# Autodesk Inventor assembly: Assembly33
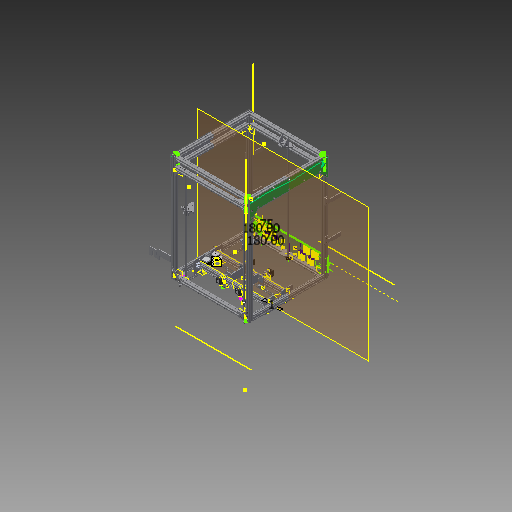
[picture p0: Inventor's stored thumbnail of the model, 512x512]
Saved by Autodesk Inventor 2018 (Build 220112000, 112)
## iProperties
Created: 2016-08-03
Part Number: Assembly33
Document SubType Name: Assembly
Designer: User
Author: User
## Documents named in this file (51)
- C:\Users\Dan\OneDrive\SL-Inventor\The Beast v1.2 PackandGo\Workspaces\Workspace\Assembly33.iam
- C:\Users\Dan\OneDrive\SL-Inventor\The Beast v1.2 PackandGo\Workspaces\Workspace\3030 900mm.ipt
- C:\Users\Dan\OneDrive\SL-Inventor\The Beast v1.2 PackandGo\Workspaces\Workspace\3030 900mm_CPY.ipt
- C:\Users\Dan\OneDrive\SL-Inventor\The Beast v1.2 PackandGo\Workspaces\Workspace\30mm Bracket_MIR2_MIR.ipt
- C:\Users\Dan\OneDrive\SL-Inventor\The Beast v1.2 PackandGo\Workspaces\Workspace\3030bracket.iam
- C:\Users\Dan\OneDrive\SL-Inventor\The Beast v1.2 PackandGo\Workspaces\Workspace\3030bracket_MIR.iam
- C:\Users\Dan\OneDrive\SL-Inventor\The Beast v1.2 PackandGo\Workspaces\Workspace\3030bracket_MIR1.iam
- C:\Users\Dan\OneDrive\SL-Inventor\The Beast v1.2 PackandGo\Workspaces\Workspace\Assembly31.iam
- C:\Users\Dan\OneDrive\SL-Inventor\The Beast v1.2 PackandGo\Workspaces\Workspace\3030corner.iam
- C:\Users\Dan\OneDrive\SL-Inventor\The Beast v1.2 PackandGo\Workspaces\Workspace\Assembly37.iam
- C:\Users\Dan\OneDrive\SL-Inventor\The Beast v1.2 PackandGo\Workspaces\Workspace\Assembly37_MIR.iam
- C:\Users\Dan\OneDrive\SL-Inventor\The Beast v1.2 PackandGo\Workspaces\Workspace\Top-Front-BRace.iam
- C:\Users\Dan\OneDrive\SL-Inventor\The Beast v1.2 PackandGo\Workspaces\Workspace\12mmsmoothrod_CPY.iam
- C:\Users\Dan\OneDrive\SL-Inventor\The Beast v1.2 PackandGo\Workspaces\Workspace\12mmsmoothrod_CPY_MIR.iam
- C:\Users\Dan\OneDrive\SL-Inventor\The Beast v1.2 PackandGo\Workspaces\Workspace\ExtruderP1.iam
- C:\Users\Dan\OneDrive\SL-Inventor\The Beast v1.2 PackandGo\Workspaces\Workspace\3030bracket_MIR_MIR1_MIR.iam
- C:\Users\Dan\OneDrive\SL-Inventor\The Beast v1.2 PackandGo\Workspaces\Workspace\3030bracket_MIR_MIR_MIR_MIR.iam
- C:\Users\Dan\OneDrive\SL-Inventor\The Beast v1.2 PackandGo\Workspaces\Workspace\Rear Lead Screw Idler.iam
- C:\Users\Dan\OneDrive\SL-Inventor\The Beast v1.2 PackandGo\Workspaces\Workspace\Nema17.ipt
- C:\Users\Dan\OneDrive\SL-Inventor\The Beast v1.2 PackandGo\Workspaces\Workspace\en-US\ANSI B18.3.1M(6)\ANSI B18.3.1M - M3x0.5 x 10(1).ipt
- C:\Users\Dan\OneDrive\SL-Inventor\The Beast v1.2 PackandGo\Workspaces\Workspace\GT2_20tooth.ipt
- C:\Users\Dan\OneDrive\SL-Inventor\The Beast v1.2 PackandGo\Workspaces\Workspace\en-US\CNS 4480\CNS 4480 - M3 x 5.ipt
- C:\Users\Dan\OneDrive\SL-Inventor\The Beast v1.2 PackandGo\Workspaces\Workspace\Nema17_MIR.ipt
- C:\Users\Dan\OneDrive\SL-Inventor\The Beast v1.2 PackandGo\Workspaces\Workspace\GT2_20tooth_MIR.ipt
- C:\Users\Dan\OneDrive\SL-Inventor\The Beast v1.2 PackandGo\Workspaces\Workspace\Side Y Rails.iam
- C:\Users\Dan\OneDrive\SL-Inventor\The Beast v1.2 PackandGo\Workspaces\Workspace\en-US\ANSI B18.3.1M(6)\ANSI B18.3.1M - M5x0.8 x 12(1).ipt
- C:\Users\Dan\OneDrive\SL-Inventor\The Beast v1.2 PackandGo\Workspaces\Workspace\M5 Tee Nut-Generic_MIR_CPY.ipt
- C:\Users\Dan\OneDrive\SL-Inventor\The Beast v1.2 PackandGo\Workspaces\Workspace\M5 Tee Nut-Generic_MIR_CPY_MIR1.ipt
- C:\Users\Dan\OneDrive\SL-Inventor\The Beast v1.2 PackandGo\Workspaces\Workspace\Front-Bed-Holder.iam
- C:\Users\Dan\OneDrive\SL-Inventor\The Beast v1.2 PackandGo\Workspaces\Workspace\Front-Bed-Holder_MIR.iam
- C:\Users\Dan\OneDrive\SL-Inventor\The Beast v1.2 PackandGo\Workspaces\Workspace\x-aXIS-aSSEMBLY.iam
- C:\Users\Dan\OneDrive\SL-Inventor\The Beast v1.2 PackandGo\Workspaces\Workspace\x-aXIS-aSSEMBLY_MIR2.iam
- C:\Users\Dan\OneDrive\SL-Inventor\The Beast v1.2 PackandGo\Workspaces\Workspace\X Axis Brace.ipt
- C:\Users\Dan\OneDrive\SL-Inventor\The Beast v1.2 PackandGo\Workspaces\Workspace\X Axis Brace_MIR.ipt
- C:\Users\Dan\OneDrive\SL-Inventor\The Beast v1.2 PackandGo\Workspaces\Workspace\en-US\ANSI B18.3.1M(6)\ANSI B18.3.1M - M3x0.5 x 16(1).ipt
- C:\Users\Dan\OneDrive\SL-Inventor\The Beast v1.2 PackandGo\Workspaces\Workspace\en-US\CSN EN 24 036\CSN EN 24 036 - M3.ipt
- C:\Users\Dan\OneDrive\SL-Inventor\The Beast v1.2 PackandGo\Workspaces\Workspace\XBELT.ipt
- C:\Users\Dan\OneDrive\SL-Inventor\The Beast v1.2 PackandGo\Workspaces\Workspace\Ziptie.ipt
- C:\Users\Dan\OneDrive\SL-Inventor\The Beast v1.2 PackandGo\Workspaces\Workspace\Ziptie_MIR.ipt
- C:\Users\Dan\OneDrive\SL-Inventor\The Beast v1.2 PackandGo\Workspaces\Workspace\YBELT.ipt
- C:\Users\Dan\OneDrive\SL-Inventor\The Beast v1.2 PackandGo\Workspaces\Workspace\YBELT_MIR.ipt
- C:\Users\Dan\OneDrive\SL-Inventor\The Beast v1.2 PackandGo\Workspaces\Workspace\handyDandy.ipt
- C:\Users\Dan\OneDrive\SL-Inventor\The Beast v1.2 PackandGo\Workspaces\Workspace\3030bracket_MIR_MIR1_MIR_MIR.iam
- C:\Users\Dan\OneDrive\SL-Inventor\The Beast v1.2 PackandGo\Workspaces\Workspace\3030bracket_MIR_MIR_MIR.iam
- C:\Users\Dan\OneDrive\SL-Inventor\The Beast v1.2 PackandGo\Workspaces\Workspace\SidePanel2.iam
- C:\Users\Dan\OneDrive\SL-Inventor\The Beast v1.2 PackandGo\Workspaces\Workspace\Front Brace.ipt
- C:\Users\Dan\OneDrive\SL-Inventor\The Beast v1.2 PackandGo\Workspaces\Workspace\BoltandTee.iam
- C:\Users\Dan\OneDrive\SL-Inventor\The Beast v1.2 PackandGo\Workspaces\Workspace\Z Endstop.iam
- C:\Users\Dan\OneDrive\SL-Inventor\The Beast v1.2 PackandGo\Workspaces\Workspace\Z Motor Mount Right.ipt
- C:\Autodesk\SL-Inventor\The Beast V2 Current PacknGo for Product Renderings\Workspaces\Workspace\Ball Bearing F608ZZ.ipt
- C:\Users\Dan\OneDrive\SL-Inventor\The Beast v1.2 PackandGo\Workspaces\Workspace\F608Brace.ipt
## Components (105 placed, 51 different names)
1. 3030 900mm:1 — Flush:65, Flush:66, Mate:107, Mate:108
2. 3030 900mm_CPY:1
3. 3030 900mm_CPY:2
4. 30mm Bracket_MIR2_MIR:1
5. 3030bracket:1 [sub-assembly]
6. 3030bracket:2 [sub-assembly]
7. X Axis Brace_MIR:1 — Mate:102, Mate:103, Flush:67
8. X Axis Brace:1
9. Forged Socket Head Cap Screw - Metric M3x0.5 x 16:1
10. Forged Socket Head Cap Screw - Metric M3x0.5 x 16:4
11. Front Brace:2
12. Front Brace:1
13. BoltandTee:10 [sub-assembly]
14. BoltandTee:9 [sub-assembly]
15. BoltandTee:8 [sub-assembly]
16. BoltandTee:7 [sub-assembly]
17. BoltandTee:6 [sub-assembly]
18. BoltandTee:5 [sub-assembly]
19. BoltandTee:4 [sub-assembly]
20. BoltandTee:3 [sub-assembly]
21. BoltandTee:2 [sub-assembly]
22. BoltandTee:1 [sub-assembly]
23. Forged Socket Head Cap Screw - Metric M3x0.5 x 16:6
24. Forged Socket Head Cap Screw - Metric M3x0.5 x 16:8
25. CSN EN 24036 M3:5
26. CSN EN 24036 M3:6
27. CSN EN 24036 M3:7
28. CSN EN 24036 M3:8
29. Forged Socket Head Cap Screw - Metric M3x0.5 x 16:5
30. Forged Socket Head Cap Screw - Metric M3x0.5 x 16:7
31. CSN EN 24036 M3:2
32. CSN EN 24036 M3:3 — Mate:97, Flush:61
33. CSN EN 24036 M3:4 — Mate:98, Flush:61
34. Forged Socket Head Cap Screw - Metric M3x0.5 x 16:3 — Mate:98
35. Forged Socket Head Cap Screw - Metric M3x0.5 x 16:2 — Mate:97
36. CSN EN 24036 M3:1
37. 3030bracket_MIR:1 [sub-assembly]
38. 3030bracket_MIR:2 [sub-assembly]
39. 3030bracket_MIR1:1 [sub-assembly]
40. 3030bracket_MIR1:2 [sub-assembly]
41. Assembly31:1 [sub-assembly] — Mate:73, Flush:58, Mate:101, Mate:106
42. SpoolHolder [sub-assembly]
43. Assembly37:2 [sub-assembly]
44. Assembly37_MIR:1 [sub-assembly]
45. Assembly37_MIR:2 [sub-assembly]
46. Top-Front-BRace:1 [sub-assembly]
47. 3030corner:1 [sub-assembly] — Mate:100, Flush:63, Flush:64
48. 12mmsmoothrod_CPY:1 [sub-assembly]
49. 12mmsmoothrod_CPY_MIR:1 [sub-assembly]
50. 3030bracket_MIR_MIR1_MIR:1 [sub-assembly]
51. Side Y Rails:1 [sub-assembly]
52. 3030bracket_MIR_MIR_MIR_MIR:1 [sub-assembly]
53. Front-Bed-Holder:1 [sub-assembly]
54. Front-Bed-Holder_MIR:1 [sub-assembly]
55. YBELT_MIR:1
56. YBELT:1
57. ExtruderP1:1 [sub-assembly] — Flush:62
58. Nema17_MIR:1
59. M5 Tee Nut-Generic_MIR_CPY:3
60. M5 Tee Nut-Generic_MIR_CPY:4
61. x-aXIS-aSSEMBLY:1 [sub-assembly]
62. Forged Socket Head Cap Screw - Metric M5x0.8 x 12:3
63. M5 Tee Nut-Generic_MIR_CPY:2
64. Forged Socket Head Cap Screw - Metric M5x0.8 x 12:1
65. M5 Tee Nut-Generic_MIR_CPY:1
66. M5 Tee Nut-Generic_MIR_CPY_MIR1:3
67. M5 Tee Nut-Generic_MIR_CPY_MIR1:4
68. M5 Tee Nut-Generic_MIR_CPY_MIR1:1
69. M5 Tee Nut-Generic_MIR_CPY_MIR1:2
70. Forged Socket Head Cap Screw - Metric M3x0.5 x 10:7
71. Forged Socket Head Cap Screw - Metric M3x0.5 x 10:5
72. Forged Socket Head Cap Screw - Metric M3x0.5 x 10:6
73. Forged Socket Head Cap Screw - Metric M3x0.5 x 10:8
74. GT2_20tooth_MIR:1
75. Nema17:1
76. Forged Socket Head Cap Screw - Metric M3x0.5 x 10:1
77. Forged Socket Head Cap Screw - Metric M3x0.5 x 10:2
78. Forged Socket Head Cap Screw - Metric M3x0.5 x 10:4
79. Forged Socket Head Cap Screw - Metric M3x0.5 x 10:3
80. GT2_20tooth:1
81. CNS 4480 M3 x 5:2
82. CNS 4480 M3 x 5:1
83. CNS 4480 M3 x 5:4
84. CNS 4480 M3 x 5:3
85. Rear Lead Screw Idler:1 [sub-assembly]
86. 12mmsmoothrod_CPY_MIR:2 [sub-assembly] — Mate:73, Flush:58
87. XBELT:1
88. x-aXIS-aSSEMBLY_MIR2:1 [sub-assembly] — Mate:102, Mate:103, Flush:67
89. Ziptie:1
90. Ziptie:2
91. Ziptie_MIR:1
92. Ziptie_MIR:2
93. Ziptie_MIR:3
94. Ziptie_MIR:4
95. Ziptie_MIR:5
96. Ziptie_MIR:6
97. handyDandy:1
98. 3030bracket_MIR_MIR1_MIR_MIR:1 [sub-assembly]
99. 3030bracket_MIR_MIR_MIR:1 [sub-assembly]
100. SidePanel2:1 [sub-assembly] — Mate:101, Flush:65, Flush:66
101. SidePanel2:2 [sub-assembly] — Mate:100, Flush:63, Flush:64
102. Z Endstop:1 [sub-assembly]
103. Z Motor Mount Right:1 — Mate:106, Mate:107, Mate:108, Flush:72
104. Ball Bearing F608ZZ:1 — Mate:109, Mate:110
105. F608Brace:1 — Flush:72, Mate:109, Mate:110
## Relationships (157: Mate 77, Flush 50, Insert 22, Angle 8)
- [Mate]: Assembly31:1 ↔ 3030corner:1
- [Mate]: Assembly31:1 ↔ 3030corner:1
- [Flush] (-0.958 mm): Assembly31:1 ↔ 3030corner:1
- [Flush]: 3030 900mm:1 ↔ Assembly31:1
- [Flush]: Assembly31:1 ↔ 3030corner:1
- [Flush]: Assembly31:1 ↔ 3030corner:1
- [Mate]: Assembly31:1 ↔ 3030corner:1
- [Mate]: Assembly31:1 ↔ 3030corner:1
- [Flush]: Assembly31:1 ↔ 3030corner:1
- [Flush]: 3030 900mm:1 ↔ Assembly31:1
- [Flush]: 3030 900mm:1 ↔ Assembly31:1
- [Mate]: 3030 900mm:1 ↔ Assembly31:1
- [Mate]: 3030 900mm:1 ↔ Assembly31:1
- [Flush]: 3030 900mm:1 ↔ Assembly31:1
- [Flush]: 3030 900mm_CPY:2 ↔ Assembly31:1
- [Flush]: 3030 900mm_CPY:1 ↔ Assembly31:1
- [Flush]: 3030 900mm_CPY:2 ↔ Assembly31:1
- [Flush]: 3030 900mm_CPY:1 ↔ Assembly31:1
- [Mate]: 3030 900mm_CPY:2 ↔ Assembly31:1
- [Mate]: 3030 900mm_CPY:1 ↔ Assembly31:1
- [Flush]: 3030 900mm_CPY:1 ↔ Assembly31:1
- [Flush]: 3030 900mm_CPY:1 ↔ Assembly31:1
- [Mate]: 3030 900mm_CPY:2 ↔ Assembly31:1
- [Mate]: 3030 900mm_CPY:2 ↔ Assembly31:1
- [Mate]: 3030 900mm_CPY:1 ↔ 3030bracket:1
- [Mate]: 3030bracket:1 ↔ Assembly31:1
- [Flush]: 3030 900mm_CPY:1 ↔ 3030bracket:1
- [Mate]: 3030bracket:1 ↔ Assembly31:1
- [Mate]: 3030 900mm_CPY:1 ↔ 3030bracket:1
- [Mate]: 3030 900mm_CPY:1 ↔ 3030bracket:2
- [Flush]: 3030 900mm_CPY:1 ↔ 3030bracket:2
- [Mate]: 3030bracket:2 ↔ Assembly31:1
- [Mate]: 3030 900mm_CPY:1 ↔ SpoolHolder
- [Flush]: 3030 900mm_CPY:1 ↔ SpoolHolder
- [Angle] (0 deg): SpoolHolder ↔ Assembly37:2
- [Mate]: 3030 900mm_CPY:1 ↔ Assembly37:2
- [Flush]: 3030 900mm_CPY:1 ↔ Assembly37:2
- [Angle] (0 deg): Assembly37_MIR:1 ↔ Assembly37_MIR:2
- [Flush]: 3030 900mm:1 ↔ Top-Front-BRace:1
- [Mate]: 3030 900mm:1 ↔ Top-Front-BRace:1
- [Flush]: 3030 900mm:1 ↔ Top-Front-BRace:1
- [Mate]: Top-Front-BRace:1 ↔ 3030corner:1
- [Mate]: Top-Front-BRace:1 ↔ 12mmsmoothrod_CPY:1
- [Mate]: Top-Front-BRace:1 ↔ 12mmsmoothrod_CPY_MIR:1
- [Flush]: 3030 900mm_CPY:1 ↔ ExtruderP1:1
- [Flush]: 3030 900mm_CPY:1 ↔ ExtruderP1:1
- [Mate]: 3030 900mm_CPY:1 ↔ ExtruderP1:1
- [Mate]: 3030 900mm_CPY:1 ↔ ExtruderP1:1
- [Flush]: 3030 900mm_CPY:1 ↔ ExtruderP1:1
- [Mate]: 3030 900mm_CPY:2 ↔ ExtruderP1:1
- [Mate]: ExtruderP1:1 ↔ Rear Lead Screw Idler:1
- [Mate]: ExtruderP1:1 ↔ Nema17:1
- [Mate]: ExtruderP1:1 ↔ Nema17:1
- [Insert]: ExtruderP1:1 ↔ Forged Socket Head Cap Screw - Metric M3x0.5 x 10:1
- [Insert]: ExtruderP1:1 ↔ Forged Socket Head Cap Screw - Metric M3x0.5 x 10:2
- [Insert]: ExtruderP1:1 ↔ Forged Socket Head Cap Screw - Metric M3x0.5 x 10:3
- [Insert]: ExtruderP1:1 ↔ Forged Socket Head Cap Screw - Metric M3x0.5 x 10:4
- [Flush]: Nema17:1 ↔ GT2_20tooth:1
- [Mate]: Nema17:1 ↔ GT2_20tooth:1
- [Mate]: GT2_20tooth:1 ↔ CNS 4480 M3 x 5:2
- [Mate]: GT2_20tooth:1 ↔ CNS 4480 M3 x 5:1
- [Mate]: ExtruderP1:1 ↔ Nema17_MIR:1
- [Mate]: ExtruderP1:1 ↔ Nema17_MIR:1
- [Insert]: ExtruderP1:1 ↔ Forged Socket Head Cap Screw - Metric M3x0.5 x 10:5
- [Insert]: ExtruderP1:1 ↔ Forged Socket Head Cap Screw - Metric M3x0.5 x 10:6
- [Insert]: ExtruderP1:1 ↔ Forged Socket Head Cap Screw - Metric M3x0.5 x 10:7
- [Insert]: ExtruderP1:1 ↔ Forged Socket Head Cap Screw - Metric M3x0.5 x 10:8
- [Mate]: Nema17_MIR:1 ↔ GT2_20tooth_MIR:1
- [Flush]: Nema17_MIR:1 ↔ GT2_20tooth_MIR:1
- [Mate]: GT2_20tooth_MIR:1 ↔ CNS 4480 M3 x 5:3
- [Mate]: GT2_20tooth_MIR:1 ↔ CNS 4480 M3 x 5:4
- [Flush]: 3030 900mm:1 ↔ Side Y Rails:1
- [Mate]: 3030 900mm:1 ↔ Side Y Rails:1
- [Flush]: Top-Front-BRace:1 ↔ Side Y Rails:1
- [Mate]: Forged Socket Head Cap Screw - Metric M5x0.8 x 12:1 ↔ M5 Tee Nut-Generic_MIR_CPY:1
- [Mate]: Forged Socket Head Cap Screw - Metric M5x0.8 x 12:3 ↔ M5 Tee Nut-Generic_MIR_CPY:2
- [Flush]: M5 Tee Nut-Generic_MIR_CPY:2 ↔ M5 Tee Nut-Generic_MIR_CPY:1
- [Flush]: M5 Tee Nut-Generic_MIR_CPY:3 ↔ M5 Tee Nut-Generic_MIR_CPY:2
- [Flush]: M5 Tee Nut-Generic_MIR_CPY:3 ↔ M5 Tee Nut-Generic_MIR_CPY:4
- [Flush] (3 mm): Assembly31:1 ↔ M5 Tee Nut-Generic_MIR_CPY:4
- [Angle] (0 deg): M5 Tee Nut-Generic_MIR_CPY:2 ↔ M5 Tee Nut-Generic_MIR_CPY:1
- [Angle] (0 deg): M5 Tee Nut-Generic_MIR_CPY:3 ↔ M5 Tee Nut-Generic_MIR_CPY:2
- [Angle] (0 deg): M5 Tee Nut-Generic_MIR_CPY:3 ↔ M5 Tee Nut-Generic_MIR_CPY:4
- [Angle] (0 deg): M5 Tee Nut-Generic_MIR_CPY_MIR1:1 ↔ M5 Tee Nut-Generic_MIR_CPY_MIR1:2
- [Flush]: M5 Tee Nut-Generic_MIR_CPY_MIR1:1 ↔ M5 Tee Nut-Generic_MIR_CPY_MIR1:2
- [Angle] (0 deg): M5 Tee Nut-Generic_MIR_CPY_MIR1:3 ↔ M5 Tee Nut-Generic_MIR_CPY_MIR1:2
- [Flush]: M5 Tee Nut-Generic_MIR_CPY_MIR1:3 ↔ M5 Tee Nut-Generic_MIR_CPY_MIR1:2
- [Angle] (0 deg): M5 Tee Nut-Generic_MIR_CPY_MIR1:3 ↔ M5 Tee Nut-Generic_MIR_CPY_MIR1:4
- [Flush]: M5 Tee Nut-Generic_MIR_CPY_MIR1:3 ↔ M5 Tee Nut-Generic_MIR_CPY_MIR1:4
- [Mate]: 12mmsmoothrod_CPY:1 ↔ Front-Bed-Holder:1
- [Flush]: Front-Bed-Holder:1 ↔ Front-Bed-Holder_MIR:1
- [Mate]: 12mmsmoothrod_CPY_MIR:1 ↔ Z Endstop:1
- Mate:73: Assembly31:1 ↔ 12mmsmoothrod_CPY_MIR:2
- Flush:58: Assembly31:1 ↔ 12mmsmoothrod_CPY_MIR:2
- [Mate]: X Axis Brace:1 ↔ x-aXIS-aSSEMBLY:1
- [Mate]: X Axis Brace:1 ↔ x-aXIS-aSSEMBLY:1
- [Flush]: X Axis Brace:1 ↔ x-aXIS-aSSEMBLY:1
- [Flush]: X Axis Brace_MIR:1 ↔ x-aXIS-aSSEMBLY:1
- [Mate]: X Axis Brace_MIR:1 ↔ x-aXIS-aSSEMBLY:1
- [Mate]: X Axis Brace_MIR:1 ↔ x-aXIS-aSSEMBLY:1
- [Insert]: X Axis Brace:1 ↔ Forged Socket Head Cap Screw - Metric M3x0.5 x 16:1
- [Insert]: X Axis Brace:1 ↔ Forged Socket Head Cap Screw - Metric M3x0.5 x 16:2
- [Insert]: X Axis Brace:1 ↔ Forged Socket Head Cap Screw - Metric M3x0.5 x 16:3
- [Insert]: X Axis Brace:1 ↔ Forged Socket Head Cap Screw - Metric M3x0.5 x 16:4
- [Mate]: X Axis Brace_MIR:1 ↔ Forged Socket Head Cap Screw - Metric M3x0.5 x 16:5
- [Mate]: X Axis Brace_MIR:1 ↔ Forged Socket Head Cap Screw - Metric M3x0.5 x 16:5
- [Mate]: X Axis Brace_MIR:1 ↔ Forged Socket Head Cap Screw - Metric M3x0.5 x 16:6
- [Mate]: X Axis Brace_MIR:1 ↔ Forged Socket Head Cap Screw - Metric M3x0.5 x 16:6
- [Mate]: X Axis Brace_MIR:1 ↔ Forged Socket Head Cap Screw - Metric M3x0.5 x 16:7
- [Mate]: X Axis Brace_MIR:1 ↔ Forged Socket Head Cap Screw - Metric M3x0.5 x 16:7
- [Mate]: X Axis Brace_MIR:1 ↔ Forged Socket Head Cap Screw - Metric M3x0.5 x 16:8
- [Mate]: X Axis Brace_MIR:1 ↔ Forged Socket Head Cap Screw - Metric M3x0.5 x 16:8
- [Mate]: Forged Socket Head Cap Screw - Metric M3x0.5 x 16:5 ↔ CSN EN 24036 M3:1
- [Mate]: Forged Socket Head Cap Screw - Metric M3x0.5 x 16:7 ↔ CSN EN 24036 M3:2
- [Mate]: CSN EN 24036 M3:4 ↔ Forged Socket Head Cap Screw - Metric M3x0.5 x 16:3
- [Mate]: Forged Socket Head Cap Screw - Metric M3x0.5 x 16:6 ↔ CSN EN 24036 M3:5
- [Mate]: CSN EN 24036 M3:5 ↔ x-aXIS-aSSEMBLY:1
- [Mate]: Forged Socket Head Cap Screw - Metric M3x0.5 x 16:8 ↔ CSN EN 24036 M3:6
- [Mate]: CSN EN 24036 M3:6 ↔ x-aXIS-aSSEMBLY:1
- [Mate]: Forged Socket Head Cap Screw - Metric M3x0.5 x 16:1 ↔ CSN EN 24036 M3:7
- [Mate]: CSN EN 24036 M3:7 ↔ x-aXIS-aSSEMBLY:1
- [Mate]: CSN EN 24036 M3:8 ↔ x-aXIS-aSSEMBLY:1
- Mate:97: CSN EN 24036 M3:3 ↔ Forged Socket Head Cap Screw - Metric M3x0.5 x 16:2
- Mate:98: CSN EN 24036 M3:4 ↔ Forged Socket Head Cap Screw - Metric M3x0.5 x 16:3
- Flush:61: CSN EN 24036 M3:3 ↔ CSN EN 24036 M3:4
- Flush:62 (300 mm): ExtruderP1:1
- Mate:100: 3030corner:1 ↔ SidePanel2:2
- Flush:63: 3030corner:1 ↔ SidePanel2:2
- Flush:64: 3030corner:1 ↔ SidePanel2:2
- Mate:101: Assembly31:1 ↔ SidePanel2:1
- Flush:65: 3030 900mm:1 ↔ SidePanel2:1
- Flush:66: 3030 900mm:1 ↔ SidePanel2:1
- Mate:102: X Axis Brace_MIR:1 ↔ x-aXIS-aSSEMBLY_MIR2:1
- Mate:103: X Axis Brace_MIR:1 ↔ x-aXIS-aSSEMBLY_MIR2:1
- Flush:67: X Axis Brace_MIR:1 ↔ x-aXIS-aSSEMBLY_MIR2:1
- [Mate]: Front Brace:1 ↔ 3030corner:1
- [Flush]: Front Brace:1 ↔ 3030corner:1
- [Flush]: Front Brace:1 ↔ Top-Front-BRace:1
- [Mate]: 3030 900mm:1 ↔ Front Brace:2
- [Flush]: Front Brace:2 ↔ Top-Front-BRace:1
- [Flush]: 3030 900mm:1 ↔ Front Brace:2
- [Insert]: Front Brace:2 ↔ BoltandTee:5
- [Insert]: Front Brace:2 ↔ BoltandTee:4
- [Insert]: Front Brace:2 ↔ BoltandTee:3
- [Insert]: Front Brace:2 ↔ BoltandTee:2
- [Insert]: Front Brace:2 ↔ BoltandTee:1
- [Insert]: Front Brace:1 ↔ BoltandTee:6
- [Insert]: Front Brace:1 ↔ BoltandTee:7
- [Insert]: Front Brace:1 ↔ BoltandTee:8
- [Insert]: Front Brace:1 ↔ BoltandTee:9
- [Insert]: Front Brace:1 ↔ BoltandTee:10
- Mate:106: Assembly31:1 ↔ Z Motor Mount Right:1
- Mate:107: 3030 900mm:1 ↔ Z Motor Mount Right:1
- Mate:108: 3030 900mm:1 ↔ Z Motor Mount Right:1
- Flush:72: Z Motor Mount Right:1 ↔ F608Brace:1
- Mate:109: Ball Bearing F608ZZ:1 ↔ F608Brace:1
- Mate:110: Ball Bearing F608ZZ:1 ↔ F608Brace:1
## Named parameters: d17_d36 = 0 mm, d18_d37 = 0 mm, d83_d68 = 0 mm, d84_d69 = 0 mm, d208_d23 = 0 mm
